# Autodesk Inventor assembly: Caja motriz 2b_CasaCentral
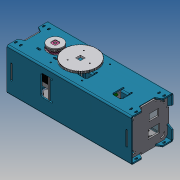
[picture p0: Inventor's stored thumbnail of the model, 180x180]
Saved by Autodesk Inventor 2017 (Build 210142000, 142)
## iProperties
Part Number: Caja motriz 2b_CasaCentral
Material: Genérico
Document SubType Name: Assembly
Designer: leo
Author: FABLAB
## Documents named in this file (8)
- C:\Users\Leo\Documents\GitHub\actor-re-actor\models\inventor-caja\Caja motriz 2b_CasaCentral.iam
- C:\Users\Leo\Documents\GitHub\actor-re-actor\models\inventor-caja\ensamble caja motriz\Design Accelerator\Conexión por perno1.iam
- C:\Users\Leo\Documents\GitHub\actor-re-actor\models\inventor-caja\ensamble caja motriz\Design Accelerator\Conexión por perno2.iam
- C:\Users\Leo\Documents\GitHub\actor-re-actor\models\inventor-caja\Piezas\componentes.iam
- C:\Users\Leo\Documents\GitHub\actor-re-actor\models\inventor-caja\Case\Case-D.iam
- C:\Users\Leo\Documents\GitHub\actor-re-actor\models\inventor-caja\Piezas\motor y golillas.iam
- C:\Users\Leo\Documents\GitHub\actor-re-actor\models\inventor-caja\partes transmision\Conjunto polea motor 2.iam
- C:\Users\Leo\Documents\GitHub\actor-re-actor\models\inventor-caja\partes transmision\conjunto polea sinfin.iam
## Components (7 placed, 6 different names)
1. Case-D:1 [sub-assembly] — Coincidencia:1, Coincidencia:9, Nivelación:12, Coincidencia:11, Coincidencia:12, Coincidencia:13, Nivelación:13, Coincidencia:14
2. motor y golillas:1 [sub-assembly] — Coincidencia:1, Coincidencia:2, Coincidencia:3, Coincidencia:10, Insertar:1
3. Conexión por perno:1 [sub-assembly] — Coincidencia:12, Coincidencia:13
4. Conexión por perno:2 [sub-assembly] — Coincidencia:9, Coincidencia:10
5. componentes:1 [sub-assembly] — Nivelación:12, Coincidencia:11, Nivelación:13
6. Conjunto polea motor 2:1 [sub-assembly] — Insertar:1
7. conjunto polea sinfin:1 [sub-assembly] — Coincidencia:14
## Relationships (12: Mate 9, Flush 2, Insert 1)
- Coincidencia:1 [Mate]: Case-D:1 ↔ motor y golillas:1
- Coincidencia:2 [Mate]: motor y golillas:1
- Coincidencia:3 [Mate]: motor y golillas:1
- Coincidencia:9 [Mate]: Case-D:1 ↔ Conexión por perno:2
- Coincidencia:10 [Mate]: motor y golillas:1 ↔ Conexión por perno:2
- Nivelación:12 [Flush]: Case-D:1 ↔ componentes:1
- Coincidencia:11 [Mate]: Case-D:1 ↔ componentes:1
- Coincidencia:12 [Mate]: Case-D:1 ↔ Conexión por perno:1
- Coincidencia:13 [Mate]: Case-D:1 ↔ Conexión por perno:1
- Nivelación:13 [Flush]: Case-D:1 ↔ componentes:1
- Insertar:1: motor y golillas:1 ↔ Conjunto polea motor 2:1
- Coincidencia:14 [Mate]: Case-D:1 ↔ conjunto polea sinfin:1
